# Autodesk Inventor assembly: TNS-assembly
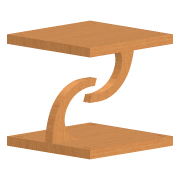
[picture p0: Inventor's stored thumbnail of the model, 180x180]
Saved by Autodesk Inventor 2020 (Build 240168000, 168)
## iProperties
Created: 2021-06-28
Part Number: TNS-assembly
Document SubType Name: Assembly
Designer: Aidan Lee
Author: Aidan Lee
## Documents named in this file (4)
- C:\Users\hobly\Dropbox\Aidan Lee\Mechanics_Walk\Tensegrity\TNS-assembly.iam
- C:\Users\hobly\Dropbox\Aidan Lee\Mechanics_Walk\Tensegrity\TNS-1-arm.ipt
- C:\Users\hobly\Dropbox\Aidan Lee\Mechanics_Walk\Tensegrity\TNS-1-platform.ipt
- C:\Users\hobly\Dropbox\Aidan Lee\Mechanics_Walk\Tensegrity\TNS-3-cover.ipt
## Components (12 placed, 3 different names)
1. TNS-1-arm:1 — Mate:12, Mate:13, Mate:14
2. TNS-1-platform:1 — Mate:12, Mate:13, Mate:14, Flush:17, Flush:18, Flush:19, Flush:20, Mate:15, Mate:23, Mate:24, Mate:25, Mate:26, Mate:27, Mate:28, Mate:29
3. TNS-1-arm:2 — Mate:1, Mate:2, Mate:3
4. TNS-1-platform:2 — Mate:1, Mate:2, Mate:3, Flush:17, Flush:18, Mate:16, Flush:21, Flush:22, Flush:23, Mate:17, Mate:18, Mate:19, Mate:20, Mate:21, Mate:22, Mate:29
5. TNS-3-cover:7 — Mate:16, Flush:21, Flush:22
6. TNS-3-cover:10 — Flush:19, Flush:20, Mate:15
7. TNS-3-cover:11 — Flush:23, Mate:17, Mate:18
8. TNS-3-cover:12 — Mate:19, Mate:20
9. TNS-3-cover:13 — Mate:21, Mate:22
10. TNS-3-cover:14 — Mate:23, Mate:24
11. TNS-3-cover:15 — Mate:25, Mate:26
12. TNS-3-cover:16 — Mate:27, Mate:28
## Relationships (28: Mate 21, Flush 7)
- Mate:1: TNS-1-arm:2 ↔ TNS-1-platform:2
- Mate:2: TNS-1-arm:2 ↔ TNS-1-platform:2
- Mate:3: TNS-1-arm:2 ↔ TNS-1-platform:2
- Mate:12: TNS-1-arm:1 ↔ TNS-1-platform:1
- Mate:13: TNS-1-arm:1 ↔ TNS-1-platform:1
- Mate:14: TNS-1-arm:1 ↔ TNS-1-platform:1
- Flush:17: TNS-1-platform:1 ↔ TNS-1-platform:2
- Flush:18: TNS-1-platform:1 ↔ TNS-1-platform:2
- Flush:19: TNS-1-platform:1 ↔ TNS-3-cover:10
- Flush:20: TNS-1-platform:1 ↔ TNS-3-cover:10
- Mate:15: TNS-1-platform:1 ↔ TNS-3-cover:10
- Mate:16: TNS-1-platform:2 ↔ TNS-3-cover:7
- Flush:21: TNS-1-platform:2 ↔ TNS-3-cover:7
- Flush:22: TNS-1-platform:2 ↔ TNS-3-cover:7
- Flush:23: TNS-1-platform:2 ↔ TNS-3-cover:11
- Mate:17: TNS-1-platform:2 ↔ TNS-3-cover:11
- Mate:18: TNS-1-platform:2 ↔ TNS-3-cover:11
- Mate:19: TNS-1-platform:2 ↔ TNS-3-cover:12
- Mate:20: TNS-1-platform:2 ↔ TNS-3-cover:12
- Mate:21: TNS-1-platform:2 ↔ TNS-3-cover:13
- Mate:22: TNS-1-platform:2 ↔ TNS-3-cover:13
- Mate:23: TNS-1-platform:1 ↔ TNS-3-cover:14
- Mate:24: TNS-1-platform:1 ↔ TNS-3-cover:14
- Mate:25: TNS-1-platform:1 ↔ TNS-3-cover:15
- Mate:26: TNS-1-platform:1 ↔ TNS-3-cover:15
- Mate:27: TNS-1-platform:1 ↔ TNS-3-cover:16
- Mate:28: TNS-1-platform:1 ↔ TNS-3-cover:16
- Mate:29 (175 mm): TNS-1-platform:1 ↔ TNS-1-platform:2
